# Autodesk Inventor assembly: Assembly2
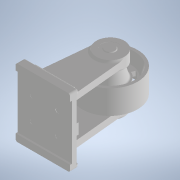
[picture p0: Inventor's stored thumbnail of the model, 180x180]
Saved by Autodesk Inventor 2021 (Build 250183000, 183)
## iProperties
Created: 2022-04-24
Part Number: Assembly2
Document SubType Name: Assembly
Designer: hp
Author: hp
## Documents named in this file (7)
- C:\Users\hp\Documents\Mechanics workspace\Inventor workspace\Homework5\Assembly2\Assembly2.iam
- C:\Users\hp\Documents\Mechanics workspace\Inventor workspace\Homework5\Assembly2\base.ipt
- C:\Users\hp\Documents\Mechanics workspace\Inventor workspace\Homework5\Assembly2\bracket.ipt
- C:\Users\hp\Documents\Mechanics workspace\Inventor workspace\Homework5\Assembly2\bushing.ipt
- C:\Users\hp\Documents\Mechanics workspace\Inventor workspace\Homework5\Assembly2\shaft.ipt
- C:\Users\hp\Documents\Mechanics workspace\Inventor workspace\Homework5\Assembly2\roller.ipt
- C:\Users\hp\Documents\Mechanics workspace\Inventor workspace\Homework5\Assembly2\connector.ipt
## Components (11 placed, 6 different names)
1. base:1 — Mate:1, Mate:2
2. bracket:1 — Mate:2, Mate:4, Mate:9, Mate:10
3. bracket:2 — Mate:1, Mate:3, Flush:1, Mate:7, Mate:8
4. bushing:1 — Mate:3, Mate:5
5. bushing:2 — Mate:4
6. shaft:1 — Mate:5, Mate:6
7. roller:1 — Mate:6
8. connector:1 — Mate:7
9. connector:2 — Mate:10
10. connector:3 — Mate:9
11. connector:4 — Mate:8
## Relationships (11: Mate 10, Flush 1)
- Mate:1: base:1 ↔ bracket:2
- Mate:2: base:1 ↔ bracket:1
- Mate:3: bracket:2 ↔ bushing:1
- Mate:4: bracket:1 ↔ bushing:2
- Mate:5: bushing:1 ↔ shaft:1
- Flush:1 (1.5 mm): bracket:2
- Mate:6: shaft:1 ↔ roller:1
- Mate:7: bracket:2 ↔ connector:1
- Mate:8: bracket:2 ↔ connector:4
- Mate:9: bracket:1 ↔ connector:3
- Mate:10: bracket:1 ↔ connector:2
